# Autodesk Inventor assembly: 207
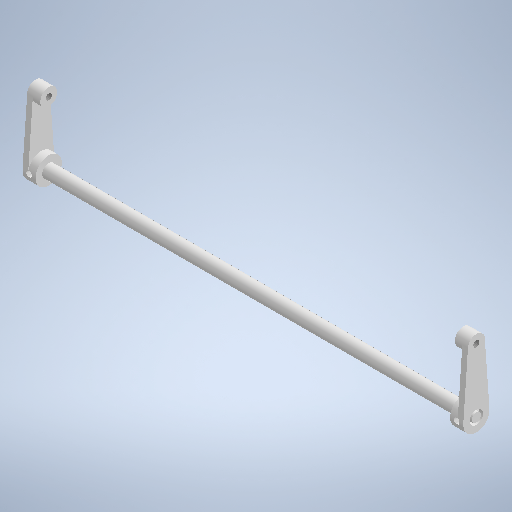
[picture p0: Inventor's stored thumbnail of the model, 512x512]
Saved by Autodesk Inventor 2025.1 (Build 291241000, 241)
## iProperties
Created: 2024-06-10
Part Number: 207
Document SubType Name: Assembly
Designer: ffogue
Author: ffogue
## Documents named in this file (3)
- C:\Users\ffogue\Downloads\Meine Projket\Paddle\207.iam
- C:\Users\ffogue\Downloads\Meine Projket\Paddle\2071.ipt
- C:\Users\ffogue\Downloads\Meine Projket\Paddle\2072.ipt
## Components (3 placed, 2 different names)
1. 2071:1 — Insert:1, Insert:2
2. 2072:1 — Insert:1
3. 2072:2 — Insert:2
## Relationships (2: Insert 2)
- Insert:1: 2071:1 ↔ 2072:1
- Insert:2: 2071:1 ↔ 2072:2
